# Autodesk Inventor assembly: MotorMountAssembly
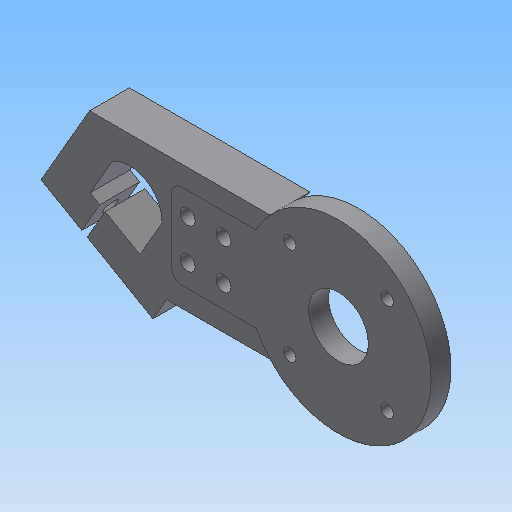
[picture p0: Inventor's stored thumbnail of the model, 512x512]
Saved by Autodesk Inventor 2017 (Build 210142000, 142)
## iProperties
Created: 2015-12-28
Part Number: MotorMountAssembly
Document SubType Name: Assembly
Designer: JoshuaYuan
Author: JoshuaYuan
## Documents named in this file (3)
- C:\Other Project Stuff\Longboard\MotorMountAssembly.iam
- C:\Other Project Stuff\Longboard\motormount3.ipt
- C:\Other Project Stuff\Longboard\motormount3_B.ipt
## Components (2 placed, 2 different names)
1. motormount3:1 — bottom mate, side mate, front mate
2. motormount3_B:1 — bottom mate, side mate, front mate
## Relationships (3: Mate 3)
- bottom mate [Mate]: motormount3:1 ↔ motormount3_B:1
- side mate [Mate]: motormount3:1 ↔ motormount3_B:1
- front mate [Mate]: motormount3:1 ↔ motormount3_B:1
